# Autodesk Inventor assembly: Робот RRO 2021
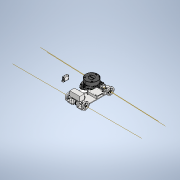
[picture p0: Inventor's stored thumbnail of the model, 180x180]
Saved by Autodesk Inventor 2020 (Build 240168000, 168)
## iProperties
Created: 2021-02-28
Part Number: Робот RRO 2021
Document SubType Name: Assembly
Designer: Антон
Author: Антон
## Documents named in this file (39)
- D:\Project\Robots\FutureEngineersViolet\3D-models\RRO 2021 Mk. IV\Робот RRO 2021 Mk. IV.iam
- D:\Project\Robots\FutureEngineersViolet\3D-models\RRO 2021 Mk. IV\Body\Основа робота.ipt
- D:\Project\Robots\FutureEngineersViolet\3D-models\RRO 2021 Mk. IV\Components\Кронштейн для двигателей серии N.ipt
- D:\Project\Robots\FutureEngineersViolet\3D-models\RRO 2021 Mk. IV\Components\Servo SG90.ipt
- D:\Project\Robots\FutureEngineersViolet\3D-models\RRO 2021 Mk. IV\Body\Основа рулевого механизма.ipt
- D:\Project\Robots\FutureEngineersViolet\3D-models\RRO 2021 Mk. IV\Components\Подшипники\Подшипник 3 8 3.ipt
- D:\Project\Robots\FutureEngineersViolet\3D-models\RRO 2021 Mk. IV\Components\Оси\Ось 3мм рулевого управления.ipt
- D:\Project\Robots\FutureEngineersViolet\3D-models\RRO 2021 Mk. IV\Body\Деталь крепления диска к поворотному механизму.ipt
- D:\Project\Robots\FutureEngineersViolet\3D-models\RRO 2021 Mk. IV\Components\Оси\Ось 3мм колеса.ipt
- D:\Project\Robots\FutureEngineersViolet\3D-models\RRO 2021 Mk. IV\Body\Деталь крепления диска к поворотному механизму_ЗЕРКАЛО1.ipt
- D:\Project\Robots\FutureEngineersViolet\3D-models\RRO 2021 Mk. IV\Components\Micro Gearmotors.ipt
- D:\Project\Robots\FutureEngineersViolet\3D-models\RRO 2021 Mk. IV\Components\Оси\Ось 2мм рулевой сервы.ipt
- D:\Project\Robots\FutureEngineersViolet\3D-models\RRO 2021 Mk. IV\Body\Поворотный рычаг для сервы.ipt
- D:\Project\Robots\FutureEngineersViolet\3D-models\RRO 2021 Mk. IV\Body\Крышка стойки подшипника 3мм.ipt
- D:\Project\Robots\FutureEngineersViolet\3D-models\RRO 2021 Mk. IV\Body\Съемная стойка сервы.ipt
- D:\Project\Robots\FutureEngineersViolet\3D-models\RRO 2021 Mk. IV\Body\Крышка поворотного кулака.ipt
- D:\Project\Robots\FutureEngineersViolet\3D-models\RRO 2021 Mk. IV\Body\Стойка подшипника 3мм.ipt
- D:\Project\Robots\FutureEngineersViolet\3D-models\RRO 2021 Mk. IV\Components\Оси\Ось 3мм задняя.ipt
- D:\Project\Robots\FutureEngineersViolet\3D-models\RRO 2021 Mk. IV\Components\Дифференциал.ipt
- D:\Project\Robots\FutureEngineersViolet\3D-models\RRO 2021 Mk. IV\Body\Ведущая шестерня дифференециала.ipt
- D:\Project\Robots\FutureEngineersViolet\3D-models\RRO 2021 Mk. IV\Components\Подшипники\Подшипник 10 15 4.ipt
- D:\Project\Robots\FutureEngineersViolet\3D-models\RRO 2021 Mk. IV\Body\Переходник с дифференциала на ось 3мм.ipt
- D:\Project\Robots\FutureEngineersViolet\3D-models\RRO 2021 Mk. IV\Components\Оси\Ось мотора серии N.ipt
- D:\Project\Robots\FutureEngineersViolet\3D-models\RRO 2021 Mk. IV\Body\Крепление дифференциала.ipt
- D:\Project\Robots\FutureEngineersViolet\3D-models\RRO 2021 Mk. IV\Body\Крепление двигателя.ipt
- D:\Project\Robots\FutureEngineersViolet\3D-models\RRO 2021 Mk. IV\Body\Проставка для двигателя.ipt
- D:\Project\Robots\FutureEngineersViolet\3D-models\RRO 2021 Mk. IV\Components\Колесо D40 под ось моторов серии N.ipt
- D:\Project\Robots\FutureEngineersViolet\3D-models\RRO 2021 Mk. IV\Body\Деталь основы рулевого управления.ipt
- D:\Project\Robots\FutureEngineersViolet\3D-models\RRO 2021 Mk. IV\Body\Крепление USB.ipt
- D:\Project\Robots\FutureEngineersViolet\3D-models\RRO 2021 Mk. IV\Body\Крышка USB.ipt
- D:\Project\Robots\FutureEngineersViolet\3D-models\RRO 2021 Mk. IV\Components\Подшипники\Подшипник 3 8 4.ipt
- D:\Project\Robots\FutureEngineersViolet\3D-models\RRO 2021 Mk. IV\Components\nVision lipo battery.ipt
- D:\Project\Robots\FutureEngineersViolet\3D-models\RRO 2021 Mk. IV\Body\Стойка под электроннику.ipt
- D:\Project\Robots\FutureEngineersViolet\3D-models\RRO 2021 Mk. IV\Body\Лого ШП.ipt
- D:\Project\Robots\FutureEngineersViolet\3D-models\RRO 2021 Mk. IV\Body\Рулевая тяга правая.ipt
- D:\Project\Robots\FutureEngineersViolet\3D-models\RRO 2021 Mk. IV\Body\Рулевая тяга левая.ipt
- D:\Project\Robots\FutureEngineersViolet\3D-models\RRO 2021 Mk. IV\Components\RPLIDAR A1M8\RPLIDAR A1M8.iam
- D:\Project\Robots\FutureEngineersViolet\3D-models\RRO 2021 Mk. IV\Test\Тестовая схема расположения электронники 2.ipt
- D:\Project\Robots\FutureEngineersViolet\3D-models\RRO 2021 Mk. IV\Test\Тестовая схема расположения электронники.ipt
## Components (61 placed, 37 different names)
1. Основа робота:1 — Жесткий:152, Жесткий:153, Жесткий:189, Жесткий:190, Жесткий:226, Жесткий:258, Жесткий:267, Жесткий:268
2. RPLIDAR A1M8:1 [sub-assembly]
3. Основа рулевого механизма:1 — Жесткий:45, Жесткий:226, Жесткий:236, Жесткий:238, С поворотом:244, С поворотом:248, Жесткий:249, Жесткий:250, Жесткий:260
4. Съемная стойка сервы:1 — Жесткий:260
5. Servo SG90:2 — С поворотом:163, Жесткий:238
6. Поворотный рычаг для сервы:1 — С поворотом:163, Жесткий:259, С поворотом:253
7. Ось 2мм рулевой сервы:1 — Жесткий:259
8. Деталь основы рулевого управления:2 — Жесткий:248, Жесткий:250
9. Рулевая тяга левая:2 — С поворотом:249, С поворотом:252
10. Деталь основы рулевого управления:1 — Жесткий:223, Жесткий:249
11. Рулевая тяга левая:1 — С поворотом:250, С поворотом:252, С поворотом:253
12. Стойка под электроннику:1 — Жесткий:241, Жесткий:262, Жесткий:267
13. Лого ШП:1 — Жесткий:241
14. Ось 3мм задняя:2 — Жесткий:165, Жесткий:197
15. Переходник с дифференциала на ось 3мм:1 — Жесткий:165, Жесткий:171
16. Крепление двигателя:1 — Жесткий:213, Жесткий:264
17. Дифференциал:1 — С поворотом:158, Жесткий:166, ЗубчПер:1, Жесткий:171, С поворотом:164
18. Переходник с дифференциала на ось 3мм:2 — Жесткий:166, Жесткий:170
19. Ось 3мм задняя:1 — Жесткий:170, Жесткий:196
20. nVision lipo battery:1 — Жесткий:262
21. Тестовая схема расположения электронники 2:1 — Жесткий:264
22. Тестовая схема расположения электронники:1
23. nVision lipo battery:2 — Жесткий:258
24. Крышка поворотного кулака:3 — Жесткий:239
25. Деталь крепления диска к поворотному механизму:1 — Жесткий:13, Жесткий:14, Жесткий:229, Жесткий:239, С поворотом:244, С поворотом:249
26. Крышка поворотного кулака:4 — Жесткий:237
27. Деталь крепления диска к поворотному механизму_ЗЕРКАЛО1:1 — Жесткий:247, Жесткий:228, Жесткий:237, Жесткий:246, С поворотом:248, С поворотом:250
28. Крышка стойки подшипника 3мм:1 — Жесткий:109, Жесткий:110
29. Подшипник 3*8*3:9 — Жесткий:109
30. Стойка подшипника 3мм:1 — Жесткий:110, Жесткий:153
31. Крепление дифференциала:1 — Жесткий:188, Жесткий:189, Жесткий:213
32. Подшипник 10 15 4:1 — С поворотом:158, Жесткий:188
33. Кронштейн для двигателей серии N:1 — Жесткий:174, Жесткий:269
34. Micro Gearmotors:1 — С поворотом:160, Жесткий:174
35. Проставка для двигателя:1 — Жесткий:268, Жесткий:269
36. Ось мотора серии N:1 — С поворотом:160, Жесткий:192
37. Ведущая шестерня дифференециала:1 — ЗубчПер:1, Жесткий:192
38. Крепление дифференциала:2 — Жесткий:190
39. Подшипник 10 15 4:2 — С поворотом:164
40. Крышка стойки подшипника 3мм:4 — Жесткий:114, Жесткий:163
41. Подшипник 3*8*3:10 — Жесткий:163
42. Стойка подшипника 3мм:4 — Жесткий:114, Жесткий:152
43. Колесо D40 под ось моторов серии N:3 — Жесткий:198
44. Колесо D40 под ось моторов серии N:2 — Жесткий:199
45. Колесо D40 под ось моторов серии N:4 — Жесткий:197
46. Колесо D40 под ось моторов серии N:1 — Жесткий:196
47. Ось 3мм рулевого управления:3 — Жесткий:14
48. Ось 3мм колеса:1 — Жесткий:199, С поворотом:166
49. Ось 3мм рулевого управления:1 — Жесткий:13
50. Подшипник 3*8*4:1 — Жесткий:229, С поворотом:167
51. Подшипник 3*8*3:2 — Жесткий:45
52. Подшипник 3*8*3:3 — Жесткий:248
53. Ось 3мм рулевого управления:4 — Жесткий:247
54. Ось 3мм колеса:2 — Жесткий:198, С поворотом:167
55. Ось 3мм рулевого управления:5 — Жесткий:246
56. Подшипник 3*8*4:2 — Жесткий:228, С поворотом:166
57. Подшипник 3*8*3:7 — Жесткий:223
58. Подшипник 3*8*3:6 — Жесткий:236
59. Крепление USB:1 — Жесткий:220
60. Крепление USB:2 — Жесткий:221
61. Крышка USB:1 — Жесткий:220, Жесткий:221
## Relationships (60: WeldJoint 47, RevoluteJoint 12, RelateRotation 1)
- Жесткий:13 [WeldJoint]: Деталь крепления диска к поворотному механизму:1 ↔ Ось 3мм рулевого управления:1
- Жесткий:14 [WeldJoint]: Деталь крепления диска к поворотному механизму:1 ↔ Ось 3мм рулевого управления:3
- Жесткий:45 [WeldJoint]: Основа рулевого механизма:1 ↔ Подшипник 3*8*3:2
- Жесткий:109 [WeldJoint] (-0.05 mm): Крышка стойки подшипника 3мм:1 ↔ Подшипник 3*8*3:9
- Жесткий:110 [WeldJoint]: Крышка стойки подшипника 3мм:1 ↔ Стойка подшипника 3мм:1
- Жесткий:114 [WeldJoint]: Крышка стойки подшипника 3мм:4 ↔ Стойка подшипника 3мм:4
- Жесткий:152 [WeldJoint]: Основа робота:1 ↔ Стойка подшипника 3мм:4
- Жесткий:153 [WeldJoint]: Основа робота:1 ↔ Стойка подшипника 3мм:1
- С поворотом:158 [RevoluteJoint] (-1 mm): Дифференциал:1 ↔ Подшипник 10 15 4:1
- Жесткий:163 [WeldJoint] (-0.05 mm): Крышка стойки подшипника 3мм:4 ↔ Подшипник 3*8*3:10
- Жесткий:165 [WeldJoint]: Ось 3мм задняя:2 ↔ Переходник с дифференциала на ось 3мм:1
- Жесткий:166 [WeldJoint]: Дифференциал:1 ↔ Переходник с дифференциала на ось 3мм:2
- Жесткий:170 [WeldJoint]: Переходник с дифференциала на ось 3мм:2 ↔ Ось 3мм задняя:1
- ЗубчПер:1 [RelateRotation] (2 ul): Дифференциал:1 ↔ Ведущая шестерня дифференециала:1
- С поворотом:160 [RevoluteJoint]: Micro Gearmotors:1 ↔ Ось мотора серии N:1
- Жесткий:171 [WeldJoint]: Переходник с дифференциала на ось 3мм:1 ↔ Дифференциал:1
- Жесткий:174 [WeldJoint]: Кронштейн для двигателей серии N:1 ↔ Micro Gearmotors:1
- С поворотом:163 [RevoluteJoint] (2 mm): Servo SG90:2 ↔ Поворотный рычаг для сервы:1
- Жесткий:188 [WeldJoint]: Крепление дифференциала:1 ↔ Подшипник 10 15 4:1
- С поворотом:164 [RevoluteJoint] (-1 mm): Дифференциал:1 ↔ Подшипник 10 15 4:2
- Жесткий:189 [WeldJoint]: Основа робота:1 ↔ Крепление дифференциала:1
- Жесткий:190 [WeldJoint]: Основа робота:1 ↔ Крепление дифференциала:2
- Жесткий:192 [WeldJoint]: Ось мотора серии N:1 ↔ Ведущая шестерня дифференециала:1
- Жесткий:196 [WeldJoint]: Ось 3мм задняя:1 ↔ Колесо D40 под ось моторов серии N:1
- Жесткий:197 [WeldJoint]: Ось 3мм задняя:2 ↔ Колесо D40 под ось моторов серии N:4
- Жесткий:198 [WeldJoint]: Колесо D40 под ось моторов серии N:3 ↔ Ось 3мм колеса:2
- Жесткий:199 [WeldJoint]: Колесо D40 под ось моторов серии N:2 ↔ Ось 3мм колеса:1
- Жесткий:213 [WeldJoint]: Крепление двигателя:1 ↔ Крепление дифференциала:1
- Жесткий:220 [WeldJoint]: Крепление USB:1 ↔ Крышка USB:1
- Жесткий:221 [WeldJoint]: Крепление USB:2 ↔ Крышка USB:1
- Жесткий:223 [WeldJoint]: Деталь основы рулевого управления:1 ↔ Подшипник 3*8*3:7
- Жесткий:247 [WeldJoint]: Деталь крепления диска к поворотному механизму_ЗЕРКАЛО1:1 ↔ Ось 3мм рулевого управления:4
- Жесткий:226 [WeldJoint]: Основа робота:1 ↔ Основа рулевого механизма:1
- Жесткий:228 [WeldJoint]: Деталь крепления диска к поворотному механизму_ЗЕРКАЛО1:1 ↔ Подшипник 3*8*4:2
- С поворотом:166 [RevoluteJoint]: Ось 3мм колеса:1 ↔ Подшипник 3*8*4:2
- Жесткий:229 [WeldJoint]: Деталь крепления диска к поворотному механизму:1 ↔ Подшипник 3*8*4:1
- С поворотом:167 [RevoluteJoint]: Подшипник 3*8*4:1 ↔ Ось 3мм колеса:2
- Жесткий:236 [WeldJoint]: Основа рулевого механизма:1 ↔ Подшипник 3*8*3:6
- Жесткий:237 [WeldJoint]: Крышка поворотного кулака:4 ↔ Деталь крепления диска к поворотному механизму_ЗЕРКАЛО1:1
- Жесткий:238 [WeldJoint]: Основа рулевого механизма:1 ↔ Servo SG90:2
- Жесткий:239 [WeldJoint]: Крышка поворотного кулака:3 ↔ Деталь крепления диска к поворотному механизму:1
- Жесткий:241 [WeldJoint]: Стойка под электроннику:1 ↔ Лого ШП:1
- С поворотом:244 [RevoluteJoint] (0.8 mm): Основа рулевого механизма:1 ↔ Деталь крепления диска к поворотному механизму:1
- Жесткий:246 [WeldJoint]: Деталь крепления диска к поворотному механизму_ЗЕРКАЛО1:1 ↔ Ось 3мм рулевого управления:5
- С поворотом:248 [RevoluteJoint] (0.8 mm): Основа рулевого механизма:1 ↔ Деталь крепления диска к поворотному механизму_ЗЕРКАЛО1:1
- Жесткий:248 [WeldJoint]: Деталь основы рулевого управления:2 ↔ Подшипник 3*8*3:3
- Жесткий:249 [WeldJoint]: Основа рулевого механизма:1 ↔ Деталь основы рулевого управления:1
- Жесткий:250 [WeldJoint]: Основа рулевого механизма:1 ↔ Деталь основы рулевого управления:2
- Жесткий:258 [WeldJoint]: Основа робота:1 ↔ nVision lipo battery:2
- С поворотом:249 [RevoluteJoint] (0.5 mm): Рулевая тяга левая:2 ↔ Деталь крепления диска к поворотному механизму:1
- С поворотом:250 [RevoluteJoint] (0.5 mm): Рулевая тяга левая:1 ↔ Деталь крепления диска к поворотному механизму_ЗЕРКАЛО1:1
- С поворотом:252 [RevoluteJoint] (0.5 mm): Рулевая тяга левая:2 ↔ Рулевая тяга левая:1
- Жесткий:259 [WeldJoint]: Поворотный рычаг для сервы:1 ↔ Ось 2мм рулевой сервы:1
- Жесткий:260 [WeldJoint]: Основа рулевого механизма:1 ↔ Съемная стойка сервы:1
- С поворотом:253 [RevoluteJoint] (0.5 mm): Поворотный рычаг для сервы:1 ↔ Рулевая тяга левая:1
- Жесткий:262 [WeldJoint]: Стойка под электроннику:1 ↔ nVision lipo battery:1
- Жесткий:264 [WeldJoint]: Крепление двигателя:1 ↔ Тестовая схема расположения электронники 2:1
- Жесткий:267 [WeldJoint]: Основа робота:1 ↔ Стойка под электроннику:1
- Жесткий:268 [WeldJoint]: Основа робота:1 ↔ Проставка для двигателя:1
- Жесткий:269 [WeldJoint]: Кронштейн для двигателей серии N:1 ↔ Проставка для двигателя:1
